# Autodesk Inventor assembly: locomotionsubsytem
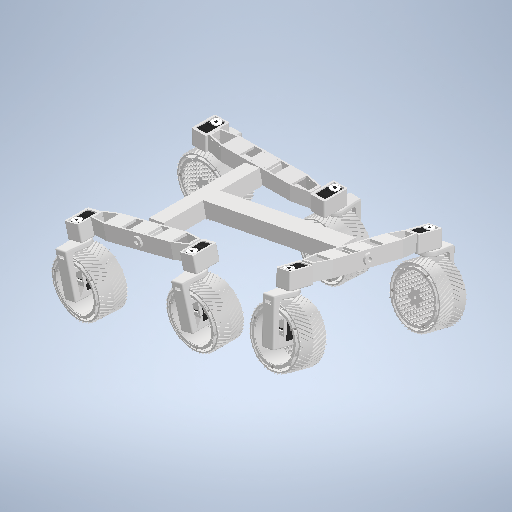
[picture p0: Inventor's stored thumbnail of the model, 512x512]
Saved by Autodesk Inventor 2025.3 (Build 293356000, 356)
## iProperties
Created: 2026-04-12
Part Number: locomotionsubsytem
Document SubType Name: Assembly
Designer: ksawe
Author: ksawe
## Documents named in this file (4)
- C:\Users\ksawe\OneDrive\Pulpit\Exomy v1\wersja2\locomotionsubsytem.iam
- C:\Users\ksawe\OneDrive\Pulpit\Exomy v1\wersja2\backpairofwheels.iam
- C:\Users\ksawe\OneDrive\Pulpit\Exomy v1\wersja2\pairofwheels.iam
- C:\Users\ksawe\OneDrive\Pulpit\Exomy v1\wersja2\T.ipt
## Components (4 placed, 3 different names)
1. backpairofwheels:1 [sub-assembly] — Mate:3, Mate:6, Mate:10
2. pairofwheels:1 [sub-assembly] — Mate:1, Mate:4, Mate:7
3. pairofwheels:2 [sub-assembly] — Mate:2, Mate:5, Mate:8, Mate:9
4. T:1 — Mate:1, Mate:2, Mate:3, Mate:4, Mate:5, Mate:6, Mate:7, Mate:8, Mate:9, Mate:10
## Relationships (10: Mate 10)
- Mate:1: pairofwheels:1 ↔ T:1
- Mate:2: pairofwheels:2 ↔ T:1
- Mate:3: backpairofwheels:1 ↔ T:1
- Mate:4: pairofwheels:1 ↔ T:1
- Mate:5: pairofwheels:2 ↔ T:1
- Mate:6: backpairofwheels:1 ↔ T:1
- Mate:7: pairofwheels:1 ↔ T:1
- Mate:8: pairofwheels:2 ↔ T:1
- Mate:9: pairofwheels:2 ↔ T:1
- Mate:10: backpairofwheels:1 ↔ T:1
